# Autodesk Inventor assembly: assembled
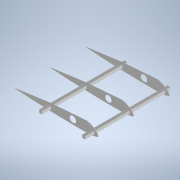
[picture p0: Inventor's stored thumbnail of the model, 180x180]
Saved by Autodesk Inventor 2021 (Build 250183000, 183)
## iProperties
Created: 2021-03-06
Part Number: assembled
Document SubType Name: Assembly
Designer: Ferdinand Hubbard
Author: Ferdinand Hubbard
## Documents named in this file (3)
- C:\Users\Ferdinand Hubbard\Desktop\solarplane\cad\right wing\right wing short.iam
- C:\Users\Ferdinand Hubbard\Desktop\solarplane\cad\airfoil.ipt
- C:\Users\Ferdinand Hubbard\Desktop\solarplane\cad\side short wood spar.ipt
## Components (5 placed, 2 different names)
1. side short wood spar:2 — Mate:2, Mate:7, Mate:10, Mate:11
2. side short wood spar:1 — Mate:1, Mate:6, Mate:9, Mate:12
3. airfoil:1 — Mate:1, Mate:2, Mate:5, Mate:11, Mate:12
4. airfoil:2 — Mate:5, Mate:6, Mate:7, Mate:8
5. airfoil:3 — Mate:8, Mate:9, Mate:10
## Relationships (10: Mate 10)
- Mate:1: side short wood spar:1 ↔ airfoil:1
- Mate:2: side short wood spar:2 ↔ airfoil:1
- Mate:5 (156.5 mm): airfoil:1 ↔ airfoil:2
- Mate:6: side short wood spar:1 ↔ airfoil:2
- Mate:7: side short wood spar:2 ↔ airfoil:2
- Mate:8 (156.5 mm): airfoil:2 ↔ airfoil:3
- Mate:9: side short wood spar:1 ↔ airfoil:3
- Mate:10: side short wood spar:2 ↔ airfoil:3
- Mate:11 (40 mm): side short wood spar:2 ↔ airfoil:1
- Mate:12 (40 mm): side short wood spar:1 ↔ airfoil:1
